# Autodesk Inventor assembly: 5 mm
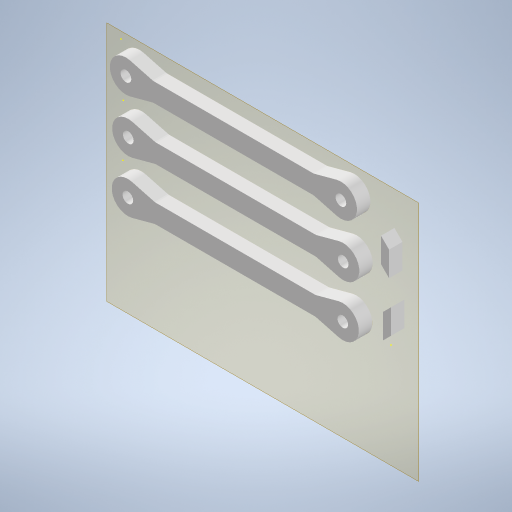
[picture p0: Inventor's stored thumbnail of the model, 512x512]
Saved by Autodesk Inventor 2023 (Build 270158000, 158)
## iProperties
Created: 2023-11-10
Part Number: 5 mm
Document SubType Name: Assembly
Designer: JULIAN
Author: JULIAN
## Documents named in this file (3)
- C:\Users\JULIAN\Desktop\Materias UN\Taller de Ingeniería Electrónica\Modelado cargo bot\DWG\5 mm.iam
- C:\Users\JULIAN\Desktop\Materias UN\Taller de Ingeniería Electrónica\Modelado cargo bot\Modelado\Mordaza.ipt
- C:\Users\JULIAN\Desktop\Materias UN\Taller de Ingeniería Electrónica\Modelado cargo bot\Modelado\Link.ipt
## Components (5 placed, 2 different names)
1. Mordaza:1 — Coincidencia:4
2. Mordaza:2 — Coincidencia:5
3. Link:1 — Coincidencia:1
4. Link:2 — Coincidencia:2
5. Link:3 — Coincidencia:3
## Relationships (5: Mate 5)
- Coincidencia:1 [Mate]: Link:1
- Coincidencia:2 [Mate]: Link:2
- Coincidencia:3 [Mate]: Link:3
- Coincidencia:4 [Mate]: Mordaza:1
- Coincidencia:5 [Mate]: Mordaza:2
